# Autodesk Inventor assembly: Assembly1
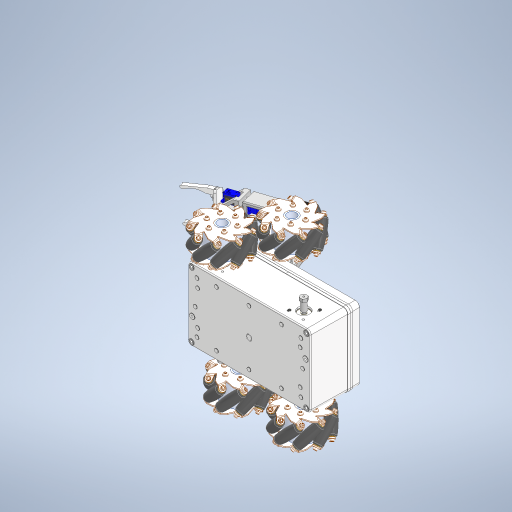
[picture p0: Inventor's stored thumbnail of the model, 512x512]
Saved by Autodesk Inventor 2024.2 (Build 282272000, 272)
## iProperties
Created: 2024-03-02
Part Number: Assembly1
Document SubType Name: Assembly
Designer: jebes windows
Author: jebes windows
## Documents named in this file (15)
- C:\Users\jebes windows\Documents\Inventor\Robotska_roka\Assembly1.iam
- C:\Users\jebes windows\Documents\Inventor\Robotska_roka\linear-gripper-1.snapshot.4\Linear Gripper\GRIPPER.iam
- C:\Users\jebes windows\Documents\Inventor\Robotska_roka\miza.ipt
- C:\Users\jebes windows\Documents\Inventor\Robotska_roka\roka3.ipt
- C:\Users\jebes windows\Documents\Inventor\Robotska_roka\roka1.ipt
- C:\Users\jebes windows\Documents\Inventor\Robotska_roka\roka2.ipt
- C:\Users\jebes windows\Documents\Inventor\Robotska_roka\sg90-micro-servo-9g-tower-pro-1.snapshot.3\SG90 - Micro Servo 9g - Tower Pro\SG90 - Micro Servo 9g - Tower Pro.iam
- C:\Users\jebes windows\Documents\Inventor\Robotska_roka\servo-motor-mg996r-1.snapshot.1(2)\Servo Motor MG996R  With Attachments\Servo Motor MG996R  With Attachments.iam
- C:\Users\jebes windows\Documents\Inventor\Robotska_roka\lemotech-ip67-junction-box-250-mm-x-150-mm-x-100-mm-1.snapshot.2\LeMotech IP67 Junction Box, 250 mm x 150 mm x 100 mm\LeMotech IP67 Junction Box, 250 mm x.iam
- C:\Users\jebes windows\Documents\Inventor\Robotska_roka\Nema 17 Motor a Pasos 17HS4401\Nema 17 Motor a Pasos 17HS4401.ipt
- C:\Users\jebes windows\Documents\Inventor\Robotska_roka\Part2.ipt
- C:\Users\jebes windows\Documents\Inventor\Robotska_roka\ArduinoMega_STEP_AP203\ArduinoMega_STEP_AP203.ipt
- C:\Users\jebes windows\Documents\Inventor\Content Center Files\R2024\en-US\DIN EN ISO 7046-2 H\DIN EN ISO 7046-2 H - M3x10 - 8.8 - H1.ipt
- C:\Users\jebes windows\Documents\Inventor\Robotska_roka\PIN.ipt
- C:\Users\jebes windows\Documents\Inventor\Robotska_roka\mecanum-wheel-diameter-100mm-right-1.snapshot.1\Mecanum Wheel (dia 100) Right\Mecanum Wheel (dia 100)\Mecanum Wheel (dia 100).ipt
## Components (37 placed, 14 different names)
1. GRIPPER:1 [sub-assembly] — Rotational:2
2. miza:1 — Insert:2, Angle:1, Mate:34, Mate:35, Mate:36
3. roka3:1 — Rotational:1, Insert:6, Angle:16
4. roka1:1 — Mate:1, Mate:2, Mate:3, Mate:4, Mate:5, Mate:6
5. roka2:1 — Insert:4, Angle:2, Insert:5, Angle:15
6. SG90 - Micro Servo 9g - Tower Pro:1 [sub-assembly] — Insert:6, Rotational:2, Angle:16
7. Servo Motor MG996R  With Attachments:1 [sub-assembly] — Insert:1, Insert:2, Angle:1
8. Servo Motor MG996R  With Attachments:2 [sub-assembly] — Insert:1, Mate:1, Mate:2, Mate:3
9. Servo Motor MG996R  With Attachments:3 [sub-assembly] — Insert:4, Angle:2
10. Servo Motor MG996R  With Attachments:4 [sub-assembly] — Mate:4, Mate:5, Mate:6
11. SG90 - Micro Servo 9g - Tower Pro:2 [sub-assembly] — Insert:5, Rotational:1, Angle:15
12. LeMotech IP67 Junction Box, 250 mm x:1 [sub-assembly] — Rigid:1, Rigid:2, Rigid:3, Rigid:4, Mate:15, Mate:16, Mate:19, Angle:9, Mate:21, Angle:10, Mate:34, Mate:35, Mate:36
13. Nema 17 Motor a Pasos 17HS4401:1 — Mate:9, Mate:10, Flush:3, Mate:18, Mate:20, Mate:24, Angle:12, Mate:28
14. Nema 17 Motor a Pasos 17HS4401:2 — Mate:7, Mate:8, Flush:4, Mate:23, Angle:13, Mate:27
15. Nema 17 Motor a Pasos 17HS4401:3 — Mate:11, Mate:12, Flush:2, Mate:22, Angle:14, Mate:26
16. Nema 17 Motor a Pasos 17HS4401:4 — Mate:13, Mate:14, Flush:1, Mate:17, Mate:25, Angle:11, Mate:29
17. Part2:1 — Rigid:3, Mate:13, Mate:14, Flush:1
18. Part2:2 — Rigid:1, Mate:9, Mate:10, Flush:3
19. Part2:3 — Rigid:2, Mate:7, Mate:8, Flush:4
20. Part2:4 — Rigid:4, Mate:11, Mate:12, Flush:2
21. ArduinoMega_STEP_AP203:1 — Mate:15, Mate:16, Mate:17
22. DIN EN ISO 7046-2 H M3x10 - 8.8 - H1:5
23. DIN EN ISO 7046-2 H M3x10 - 8.8 - H1:6
24. DIN EN ISO 7046-2 H M3x10 - 8.8 - H1:7
25. DIN EN ISO 7046-2 H M3x10 - 8.8 - H1:8
26. PIN:1 — Mate:22, Angle:14, Mate:26, Mate:32
27. PIN:2 — Mate:23, Angle:13, Mate:27
28. PIN:3 — Mate:25, Angle:11, Mate:29
29. PIN:4 — Mate:24, Angle:12, Mate:28, Mate:33
30. Mecanum Wheel (dia 100):1 — Mate:32
31. Mecanum Wheel (dia 100):2 — Mate:33
32. Mecanum Wheel (dia 100):3
33. Mecanum Wheel (dia 100):4
34. DIN EN ISO 7046-2 H M3x10 - 8.8 - H1:2 — Mate:18, Mate:19, Angle:9
35. DIN EN ISO 7046-2 H M3x10 - 8.8 - H1:1 — Mate:20, Mate:21, Angle:10
36. DIN EN ISO 7046-2 H M3x10 - 8.8 - H1:3
37. DIN EN ISO 7046-2 H M3x10 - 8.8 - H1:4
## Component patterns: (2 elements, first: DIN EN ISO 7046-2 H M3x10 - 8.8 - H1:2 + DIN EN ISO 7046-2 H M3x10 - 8.8 - H1:1)
## Relationships (60: Mate 34, Angle 10, Insert 6, WeldJoint 4, Flush 4, RevoluteJoint 2)
- Insert:1: Servo Motor MG996R  With Attachments:1 ↔ Servo Motor MG996R  With Attachments:2
- Insert:2: miza:1 ↔ Servo Motor MG996R  With Attachments:1
- Angle:1 (0 deg): miza:1 ↔ Servo Motor MG996R  With Attachments:1
- Mate:1: roka1:1 ↔ Servo Motor MG996R  With Attachments:2
- Mate:2: roka1:1 ↔ Servo Motor MG996R  With Attachments:2
- Mate:3: roka1:1 ↔ Servo Motor MG996R  With Attachments:2
- [Insert]: Servo Motor MG996R  With Attachments:3 ↔ Servo Motor MG996R  With Attachments:4
- Insert:4: roka2:1 ↔ Servo Motor MG996R  With Attachments:3
- Angle:2 (180 deg): roka2:1 ↔ Servo Motor MG996R  With Attachments:3
- Mate:4: roka1:1 ↔ Servo Motor MG996R  With Attachments:4
- Mate:5: roka1:1 ↔ Servo Motor MG996R  With Attachments:4
- Mate:6: roka1:1 ↔ Servo Motor MG996R  With Attachments:4
- Insert:5: roka2:1 ↔ SG90 - Micro Servo 9g - Tower Pro:2
- Rotational:1 [RevoluteJoint]: roka3:1 ↔ SG90 - Micro Servo 9g - Tower Pro:2
- Insert:6: roka3:1 ↔ SG90 - Micro Servo 9g - Tower Pro:1
- Rotational:2 [RevoluteJoint]: GRIPPER:1 ↔ SG90 - Micro Servo 9g - Tower Pro:1
- Rigid:1 [WeldJoint]: LeMotech IP67 Junction Box, 250 mm x:1 ↔ Part2:2
- Rigid:2 [WeldJoint]: LeMotech IP67 Junction Box, 250 mm x:1 ↔ Part2:3
- Rigid:3 [WeldJoint]: LeMotech IP67 Junction Box, 250 mm x:1 ↔ Part2:1
- Rigid:4 [WeldJoint]: LeMotech IP67 Junction Box, 250 mm x:1 ↔ Part2:4
- Mate:7: Nema 17 Motor a Pasos 17HS4401:2 ↔ Part2:3
- Mate:8: Nema 17 Motor a Pasos 17HS4401:2 ↔ Part2:3
- Mate:9: Nema 17 Motor a Pasos 17HS4401:1 ↔ Part2:2
- Mate:10: Nema 17 Motor a Pasos 17HS4401:1 ↔ Part2:2
- Mate:11: Nema 17 Motor a Pasos 17HS4401:3 ↔ Part2:4
- Mate:12: Nema 17 Motor a Pasos 17HS4401:3 ↔ Part2:4
- Mate:13: Nema 17 Motor a Pasos 17HS4401:4 ↔ Part2:1
- Mate:14: Nema 17 Motor a Pasos 17HS4401:4 ↔ Part2:1
- Flush:1: Nema 17 Motor a Pasos 17HS4401:4 ↔ Part2:1
- Flush:2: Nema 17 Motor a Pasos 17HS4401:3 ↔ Part2:4
- Flush:3: Nema 17 Motor a Pasos 17HS4401:1 ↔ Part2:2
- Flush:4: Nema 17 Motor a Pasos 17HS4401:2 ↔ Part2:3
- Mate:15: LeMotech IP67 Junction Box, 250 mm x:1 ↔ ArduinoMega_STEP_AP203:1
- Mate:16: LeMotech IP67 Junction Box, 250 mm x:1 ↔ ArduinoMega_STEP_AP203:1
- Mate:17 (3 mm): Nema 17 Motor a Pasos 17HS4401:4 ↔ ArduinoMega_STEP_AP203:1
- Mate:18: Nema 17 Motor a Pasos 17HS4401:1 ↔ DIN EN ISO 7046-2 H M3x10 - 8.8 - H1:2
- Mate:19 (0.5 mm): LeMotech IP67 Junction Box, 250 mm x:1 ↔ DIN EN ISO 7046-2 H M3x10 - 8.8 - H1:2
- Angle:9 (0 deg): LeMotech IP67 Junction Box, 250 mm x:1 ↔ DIN EN ISO 7046-2 H M3x10 - 8.8 - H1:2
- Mate:20: Nema 17 Motor a Pasos 17HS4401:1 ↔ DIN EN ISO 7046-2 H M3x10 - 8.8 - H1:1
- Mate:21 (0.5 mm): LeMotech IP67 Junction Box, 250 mm x:1 ↔ DIN EN ISO 7046-2 H M3x10 - 8.8 - H1:1
- Angle:10 (0 deg): LeMotech IP67 Junction Box, 250 mm x:1 ↔ DIN EN ISO 7046-2 H M3x10 - 8.8 - H1:1
- Mate:22: Nema 17 Motor a Pasos 17HS4401:3 ↔ PIN:1
- Mate:23: Nema 17 Motor a Pasos 17HS4401:2 ↔ PIN:2
- Mate:24: Nema 17 Motor a Pasos 17HS4401:1 ↔ PIN:4
- Mate:25: Nema 17 Motor a Pasos 17HS4401:4 ↔ PIN:3
- Angle:11 (0 deg): Nema 17 Motor a Pasos 17HS4401:4 ↔ PIN:3
- Angle:12 (0 deg): Nema 17 Motor a Pasos 17HS4401:1 ↔ PIN:4
- Angle:13 (0 deg): Nema 17 Motor a Pasos 17HS4401:2 ↔ PIN:2
- Angle:14 (0 deg): Nema 17 Motor a Pasos 17HS4401:3 ↔ PIN:1
- Mate:26: Nema 17 Motor a Pasos 17HS4401:3 ↔ PIN:1
- Mate:27: Nema 17 Motor a Pasos 17HS4401:2 ↔ PIN:2
- Mate:28: Nema 17 Motor a Pasos 17HS4401:1 ↔ PIN:4
- Mate:29: Nema 17 Motor a Pasos 17HS4401:4 ↔ PIN:3
- Mate:32: PIN:1 ↔ Mecanum Wheel (dia 100):1
- Mate:33: PIN:4 ↔ Mecanum Wheel (dia 100):2
- Mate:34: miza:1 ↔ LeMotech IP67 Junction Box, 250 mm x:1
- Mate:35: miza:1 ↔ LeMotech IP67 Junction Box, 250 mm x:1
- Mate:36: miza:1 ↔ LeMotech IP67 Junction Box, 250 mm x:1
- Angle:15 (0 deg): roka2:1 ↔ SG90 - Micro Servo 9g - Tower Pro:2
- Angle:16 (0 deg): roka3:1 ↔ SG90 - Micro Servo 9g - Tower Pro:1
## Named parameters: d7_d0 = 0 mm
